# Autodesk Inventor assembly: new design
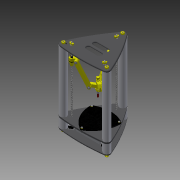
[picture p0: Inventor's stored thumbnail of the model, 180x180]
Saved by Autodesk Inventor 2013 (Build 170138000, 138)
## iProperties
Created: 2013-12-04
Part Number: new design
Document SubType Name: Assembly
Designer: employee
Author: employee
## Documents named in this file (28)
- C:\Users\employee\Desktop\ConceptFORGE\ConceptFORGE\LISA Simpson\INVENTOR FILES\LISA.iam
- C:\Users\employee\Desktop\ConceptFORGE\ConceptFORGE\LISA Simpson\INVENTOR FILES\_MID PLATE.ipt
- C:\Users\employee\Desktop\ConceptFORGE\ConceptFORGE\LISA Simpson\INVENTOR FILES\PIPE ASSEMBLY.iam
- C:\Users\employee\Desktop\ConceptFORGE\ConceptFORGE\LISA Simpson\INVENTOR FILES\_TOP PLATE.ipt
- C:\Users\employee\Desktop\ConceptFORGE\ConceptFORGE\LISA Simpson\INVENTOR FILES\_BOTTOM PLATE.ipt
- C:\Users\employee\Desktop\ConceptFORGE\ConceptFORGE\LISA Simpson\INVENTOR FILES\_STEPPER.ipt
- C:\Users\employee\Desktop\ConceptFORGE\ConceptFORGE\LISA Simpson\INVENTOR FILES\_BASALT BED.ipt
- C:\Users\employee\Desktop\ConceptFORGE\ConceptFORGE\LISA Simpson\INVENTOR FILES\THREAD ASSEMBLY.iam
- C:\Users\employee\Desktop\ConceptFORGE\ConceptFORGE\LISA Simpson\INVENTOR FILES\TENSION THREAD.iam
- C:\Users\employee\Desktop\ConceptFORGE\ConceptFORGE\LISA Simpson\INVENTOR FILES\SHOULDER.iam
- C:\Users\employee\Desktop\ConceptFORGE\ConceptFORGE\LISA Simpson\INVENTOR FILES\ARM ASSEMBLY.iam
- C:\Users\employee\Desktop\ConceptFORGE\ConceptFORGE\LISA Simpson\INVENTOR FILES\hub bottom.ipt
- C:\Users\employee\Desktop\ConceptFORGE\ConceptFORGE\LISA Simpson\INVENTOR FILES\hub center.ipt
- C:\Users\employee\Desktop\ConceptFORGE\ConceptFORGE\LISA Simpson\INVENTOR FILES\hub top.ipt
- C:\Users\employee\Desktop\ConceptFORGE\ConceptFORGE\LISA Simpson\INVENTOR FILES\_6702.ipt
- C:\Users\employee\Desktop\ConceptFORGE\ConceptFORGE\LISA Simpson\INVENTOR FILES\HUB WASHER.ipt
- C:\Users\employee\Desktop\ConceptFORGE\ConceptFORGE\LISA Simpson\INVENTOR FILES\_UBIS.ipt
- C:\Users\employee\Desktop\ConceptFORGE\ConceptFORGE\LISA Simpson\INVENTOR FILES\M8x55.ipt
- C:\Users\employee\Desktop\ConceptFORGE\ConceptFORGE\LISA Simpson\INVENTOR FILES\M8 NUT.ipt
- C:\Users\employee\Desktop\ConceptFORGE\ConceptFORGE\LISA Simpson\INVENTOR FILES\M3x20.ipt
- C:\Users\employee\Desktop\ConceptFORGE\ConceptFORGE\LISA Simpson\INVENTOR FILES\M3 NUT.ipt
- C:\Users\employee\Desktop\ConceptFORGE\ConceptFORGE\LISA Simpson\INVENTOR FILES\lock nut.ipt
- C:\Users\employee\Desktop\ConceptFORGE\ConceptFORGE\LISA Simpson\INVENTOR FILES\bowden nut.ipt
- C:\Users\employee\Desktop\ConceptFORGE\ConceptFORGE\LISA Simpson\INVENTOR FILES\PLASTIC WASHER.ipt
- C:\Users\employee\Desktop\ConceptFORGE\ConceptFORGE\LISA Simpson\INVENTOR FILES\M8x35.ipt
- C:\Users\employee\Desktop\ConceptFORGE\ConceptFORGE\LISA Simpson\INVENTOR FILES\_POWER SUPPLY.ipt
- C:\Users\employee\Desktop\ConceptFORGE\ConceptFORGE\LISA Simpson\INVENTOR FILES\STANDOFF.ipt
- C:\Users\employee\Desktop\ConceptFORGE\ConceptFORGE\LISA Simpson\INVENTOR FILES\_ELECTRONICS.ipt
## Components (55 placed, 27 different names)
1. _MID PLATE:1 — Flush:1, Mate:1, Flush:2, Insert:1, Insert:2, Insert:3, Insert:8, Insert:9, Insert:42, Insert:45, Insert:46, Insert:47
2. PIPE ASSEMBLY:1 [sub-assembly] — Insert:1, Insert:4, Insert:6
3. PIPE ASSEMBLY:2 [sub-assembly] — Insert:2, Insert:5
4. PIPE ASSEMBLY:3 [sub-assembly] — Insert:3, Insert:7
5. _TOP PLATE:1 — Insert:4, Insert:5
6. _BOTTOM PLATE:1 — Insert:6, Insert:7, Mate:2, Mate:3, Mate:4, Mate:8, Mate:11, Insert:48
7. _BASALT BED:1 — Insert:8, Insert:9, Insert:40
8. THREAD ASSEMBLY:1 [sub-assembly] — Mate:5, Mate:14, Insert:45
9. THREAD ASSEMBLY:2 [sub-assembly] — Mate:6, Mate:15, Insert:46
10. THREAD ASSEMBLY:3 [sub-assembly] — Mate:16, Insert:47
11. SHOULDER:1 [sub-assembly] — Mate:5, Insert:15, Mate:14
12. SHOULDER:2 [sub-assembly] — Mate:6, Insert:16, Mate:15
13. SHOULDER:3 [sub-assembly] — Insert:14, Mate:16
14. ARM ASSEMBLY:1 [sub-assembly] — Insert:14, Insert:25, Insert:31
15. ARM ASSEMBLY:2 [sub-assembly] — Insert:15, Insert:26, Insert:32
16. ARM ASSEMBLY:3 [sub-assembly] — Insert:16, Insert:24, Insert:33
17. hub bottom:1 — Insert:23, Insert:24, Insert:27, Insert:30, Angle:1, Angle:4, Insert:34, Insert:35, Insert:36, Insert:37, Angle:7, Angle:8, Insert:39, Angle:9, Angle:10
18. hub center:1 — Insert:17, Insert:18, Insert:25, Insert:29, Angle:3, Angle:5
19. hub top:1 — Insert:19, Insert:20, Insert:26, Insert:28, Angle:2, Angle:6
20. _6702:1 — Insert:17, Insert:23
21. _6702:2 — Insert:18, Insert:22
22. _6702:3 — Insert:20, Insert:38
23. _6702:4 — Insert:19, Insert:21
24. HUB WASHER:1 — Insert:21, Insert:22
25. _UBIS:1 — Insert:27
26. M8x55:1 — Insert:28, Angle:2
27. M8x55:2 — Insert:29, Angle:3
28. M8x55:3 — Insert:30, Angle:1
29. M8 NUT:1 — Insert:31, Angle:5
30. M8 NUT:2 — Insert:32, Angle:6
31. M8 NUT:3 — Insert:33, Angle:4
32. M3x20:1 — Insert:35
33. M3x20:2 — Insert:34
34. M3 NUT:1 — Insert:36, Angle:7
35. M3 NUT:2 — Insert:37, Angle:8
36. lock nut:1 — Insert:38, Angle:9
37. bowden nut:1 — Insert:39, Angle:10
38. _POWER SUPPLY:1 — Mate:8, Flush:3, Mate:10, Mate:12
39. STANDOFF:1 — Mate:11, Mate:12, Mate:13, Insert:43, Insert:44
40. _ELECTRONICS:1 — Insert:43, Insert:44
41. _STEPPER:1 — Mate:2, Mate:3, Mate:4
42. _STEPPER:2
43. _STEPPER:3
44. TENSION THREAD:1 [sub-assembly] — Insert:48
45. TENSION THREAD:2 [sub-assembly]
46. TENSION THREAD:3 [sub-assembly]
47. M8x35:1 — Insert:41
48. M8 NUT:4 — Insert:42
49. PLASTIC WASHER:1 — Insert:40, Insert:41
50. M8x35:2
51. M8 NUT:5
52. PLASTIC WASHER:2
53. M8x35:3
54. M8 NUT:6
55. PLASTIC WASHER:3
## Component patterns: (3 elements, first: _STEPPER:1), (3 elements, first: TENSION THREAD:1), (3 elements, first: M8x35:1 + M8 NUT:4 + PLASTIC WASHER:1)
## Relationships (71: Insert 44, Mate 14, Angle 10, Flush 3)
- Flush:1: _MID PLATE:1
- Mate:1: _MID PLATE:1
- Flush:2: _MID PLATE:1
- Insert:1: _MID PLATE:1 ↔ PIPE ASSEMBLY:1
- Insert:2: _MID PLATE:1 ↔ PIPE ASSEMBLY:2
- Insert:3: _MID PLATE:1 ↔ PIPE ASSEMBLY:3
- Insert:4: PIPE ASSEMBLY:1 ↔ _TOP PLATE:1
- Insert:5: PIPE ASSEMBLY:2 ↔ _TOP PLATE:1
- Insert:6: PIPE ASSEMBLY:1 ↔ _BOTTOM PLATE:1
- Insert:7: PIPE ASSEMBLY:3 ↔ _BOTTOM PLATE:1
- Mate:2: _BOTTOM PLATE:1 ↔ _STEPPER:1
- Mate:3: _BOTTOM PLATE:1 ↔ _STEPPER:1
- Mate:4: _BOTTOM PLATE:1 ↔ _STEPPER:1
- Insert:8: _MID PLATE:1 ↔ _BASALT BED:1
- Insert:9: _MID PLATE:1 ↔ _BASALT BED:1
- Mate:5: THREAD ASSEMBLY:1 ↔ SHOULDER:1
- Mate:6: THREAD ASSEMBLY:2 ↔ SHOULDER:2
- Insert:14: SHOULDER:3 ↔ ARM ASSEMBLY:1
- Insert:15: SHOULDER:1 ↔ ARM ASSEMBLY:2
- Insert:16: SHOULDER:2 ↔ ARM ASSEMBLY:3
- Insert:17: hub center:1 ↔ _6702:1
- Insert:18: hub center:1 ↔ _6702:2
- Insert:19: hub top:1 ↔ _6702:4
- Insert:20: hub top:1 ↔ _6702:3
- Insert:21: _6702:4 ↔ HUB WASHER:1
- Insert:22: _6702:2 ↔ HUB WASHER:1
- Insert:23: hub bottom:1 ↔ _6702:1
- Insert:24: ARM ASSEMBLY:3 ↔ hub bottom:1
- Insert:25: ARM ASSEMBLY:1 ↔ hub center:1
- Insert:26: ARM ASSEMBLY:2 ↔ hub top:1
- Insert:27: hub bottom:1 ↔ _UBIS:1
- Insert:28: hub top:1 ↔ M8x55:1
- Insert:29: hub center:1 ↔ M8x55:2
- Insert:30: hub bottom:1 ↔ M8x55:3
- Angle:1 (0 deg): hub bottom:1 ↔ M8x55:3
- Angle:2 (0 deg): hub top:1 ↔ M8x55:1
- Angle:3 (0 deg): hub center:1 ↔ M8x55:2
- Insert:31: ARM ASSEMBLY:1 ↔ M8 NUT:1
- Insert:32: ARM ASSEMBLY:2 ↔ M8 NUT:2
- Insert:33: ARM ASSEMBLY:3 ↔ M8 NUT:3
- Angle:4 (0 deg): hub bottom:1 ↔ M8 NUT:3
- Angle:5 (0 deg): hub center:1 ↔ M8 NUT:1
- Angle:6 (0 deg): hub top:1 ↔ M8 NUT:2
- Insert:34: hub bottom:1 ↔ M3x20:2
- Insert:35: hub bottom:1 ↔ M3x20:1
- Insert:36: hub bottom:1 ↔ M3 NUT:1
- Insert:37: hub bottom:1 ↔ M3 NUT:2
- Angle:7 (0 deg): hub bottom:1 ↔ M3 NUT:1
- Angle:8 (0 deg): hub bottom:1 ↔ M3 NUT:2
- Insert:38: _6702:3 ↔ lock nut:1
- Insert:39: hub bottom:1 ↔ bowden nut:1
- Angle:9 (0 deg): hub bottom:1 ↔ lock nut:1
- Angle:10 (15 deg): hub bottom:1 ↔ bowden nut:1
- Insert:40: _BASALT BED:1 ↔ PLASTIC WASHER:1
- Insert:41: M8x35:1 ↔ PLASTIC WASHER:1
- Insert:42: _MID PLATE:1 ↔ M8 NUT:4
- Mate:8: _BOTTOM PLATE:1 ↔ _POWER SUPPLY:1
- Flush:3 (88.9 mm): _POWER SUPPLY:1
- Mate:10 (-107.5055 mm): _POWER SUPPLY:1
- Mate:11: _BOTTOM PLATE:1 ↔ STANDOFF:1
- Mate:12 (44.45 mm): _POWER SUPPLY:1 ↔ STANDOFF:1
- Mate:13 (-48.3362 mm): STANDOFF:1
- Mate:14: THREAD ASSEMBLY:1 ↔ SHOULDER:1
- Mate:15: THREAD ASSEMBLY:2 ↔ SHOULDER:2
- Mate:16: THREAD ASSEMBLY:3 ↔ SHOULDER:3
- Insert:43: STANDOFF:1 ↔ _ELECTRONICS:1
- Insert:44: STANDOFF:1 ↔ _ELECTRONICS:1
- Insert:45: _MID PLATE:1 ↔ THREAD ASSEMBLY:1
- Insert:46: _MID PLATE:1 ↔ THREAD ASSEMBLY:2
- Insert:47: _MID PLATE:1 ↔ THREAD ASSEMBLY:3
- Insert:48: _BOTTOM PLATE:1 ↔ TENSION THREAD:1
